# Autodesk Inventor assembly: SubAssembly - EntireLandingSystem
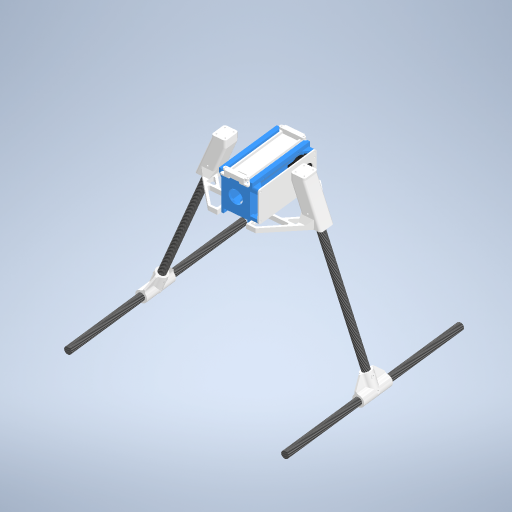
[picture p0: Inventor's stored thumbnail of the model, 512x512]
Saved by Autodesk Inventor 2023 (Build 270158000, 158)
## iProperties
Created: 2023-01-22
Part Number: SubAssembly - EntireLandingSystem
Document SubType Name: Assembly
Designer: Administrator
Author: Administrator
## Documents named in this file (3)
- C:\Users\Administrator\Documents\GitHub\WU-Team20-AutonomousDrone\CAD\ASSEMBLY\SubAssembly - EntireLandingSystem.iam
- C:\Users\Administrator\Documents\GitHub\WU-Team20-AutonomousDrone\CAD\ASSEMBLY\SubAssembly - Leg SingleSide.iam
- C:\Users\Administrator\Documents\GitHub\WU-Team20-AutonomousDrone\CAD\ASSEMBLY\SubAssembly - BatteryCarrier WithAccessories.iam
## Components (3 placed, 2 different names)
1. SubAssembly - Leg SingleSide:1 [sub-assembly] — Rigid:2
2. SubAssembly - Leg SingleSide:2 [sub-assembly] — Rigid:3
3. SubAssembly - BatteryCarrier WithAccessories:1 [sub-assembly] — Rigid:2, Rigid:3
## Relationships (2: WeldJoint 2)
- Rigid:2 [WeldJoint]: SubAssembly - Leg SingleSide:1 ↔ SubAssembly - BatteryCarrier WithAccessories:1
- Rigid:3 [WeldJoint]: SubAssembly - Leg SingleSide:2 ↔ SubAssembly - BatteryCarrier WithAccessories:1
